# Autodesk Inventor assembly: PS20025
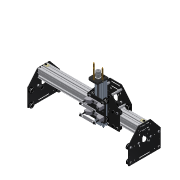
[picture p0: Inventor's stored thumbnail of the model, 180x180]
Saved by Autodesk Inventor 2014 (Build 180170000, 170)
## iProperties
Created: 2013-09-18
Part Number: PS20025
Document SubType Name: Assembly
Designer: Edward
Description: Complete Gantry
Author: Edward
Title: Complete Gantry
Subject: Shapeoko 2
## Documents named in this file (9)
- C:\Users\Edward\Documents\GitHub\Shapeoko_2\Autodesk_Inventor_Project\PS20025.iam
- C:\Users\Edward\Documents\GitHub\Shapeoko_2\Autodesk_Inventor_Project\PS20031.iam
- C:\Users\Edward\Documents\GitHub\Shapeoko_2\Autodesk_Inventor_Project\PS20008.ipt
- C:\Users\Edward\Documents\GitHub\Shapeoko_2\Autodesk_Inventor_Project\PS20022.iam
- C:\Users\Edward\Documents\GitHub\Shapeoko_2\Autodesk_Inventor_Project\25286-02.ipt
- C:\Users\Edward\Documents\GitHub\Shapeoko_2\Autodesk_Inventor_Project\25287-02.ipt
- C:\Users\Edward\Documents\GitHub\Shapeoko_2\Autodesk_Inventor_Project\26051-01.ipt
- C:\Users\Edward\Documents\GitHub\Shapeoko_2\Autodesk_Inventor_Project\PS20003.ipt
- C:\Users\Edward\Documents\GitHub\Shapeoko_2\Autodesk_Inventor_Project\26016-01.ipt
## Components (29 placed, 8 different names)
1. PS20031:1 [sub-assembly] — Mate:1, Flush:1, Mate:2, Flush:2
2. PS20022:2 [sub-assembly] — Insert:2, Insert:3, Mate:10
3. PS20008:2 — Mate:1, Flush:1, Flush:3, Insert:2, Insert:3, Mate:3, Insert:4, Insert:5, Insert:6, Insert:10, Insert:14, Insert:16
4. 25286-02:1
5. 25287-02:1 — Insert:6
6. PS20008:3 — Mate:2, Flush:2, Flush:3, Insert:11, Insert:12, Insert:18, Insert:20, Mate:7, Mate:9
7. PS20022:3 [sub-assembly] — Mate:3, Insert:4, Insert:5, Mate:8
8. 25286-02:2
9. 25287-02:2 — Insert:12
10. 25286-02:3
11. 25287-02:3 — Insert:11
12. 25286-02:4
13. 25287-02:4 — Insert:10
14. 25286-02:5
15. 25287-02:5 — Insert:14
16. 25286-02:6
17. 25287-02:6 — Insert:16
18. 25286-02:7
19. 25287-02:7 — Insert:18
20. 25286-02:8
21. 25287-02:8 — Insert:20
22. 26051-01:1 — Mate:7, Mate:8
23. PS20003:1
24. 25287-02:9
25. 26016-01:1
26. 26051-01:2 — Mate:9, Mate:10
27. PS20003:2
28. 25287-02:10
29. 26016-01:2
## Relationships (38: Insert 26, Mate 7, Flush 3, Angle 2)
- [Insert]: 25286-02:1 ↔ 25287-02:1
- Mate:1 (6.35 mm): PS20031:1 ↔ PS20008:2
- Flush:1 (25 mm): PS20031:1 ↔ PS20008:2
- Mate:2 (6.35 mm): PS20031:1 ↔ PS20008:3
- Flush:2 (25 mm): PS20031:1 ↔ PS20008:3
- Flush:3: PS20008:2 ↔ PS20008:3
- Insert:2: PS20022:2 ↔ PS20008:2
- Insert:3: PS20022:2 ↔ PS20008:2
- Mate:3: PS20008:2 ↔ PS20022:3
- Insert:4: PS20008:2 ↔ PS20022:3
- Insert:5: PS20008:2 ↔ PS20022:3
- Insert:6 (3.4163 mm): PS20008:2 ↔ 25287-02:1
- [Insert]: 25286-02:2 ↔ 25287-02:2
- [Insert]: 25286-02:3 ↔ 25287-02:3
- [Insert]: 25286-02:4 ↔ 25287-02:4
- Insert:10 (3.4163 mm): PS20008:2 ↔ 25287-02:4
- Insert:11 (3.4163 mm): PS20008:3 ↔ 25287-02:3
- Insert:12 (3.4163 mm): PS20008:3 ↔ 25287-02:2
- [Insert]: 25286-02:5 ↔ 25287-02:5
- Insert:14 (3.4163 mm): PS20008:2 ↔ 25287-02:5
- [Insert]: 25286-02:6 ↔ 25287-02:6
- Insert:16 (3.4163 mm): PS20008:2 ↔ 25287-02:6
- [Insert]: 25286-02:7 ↔ 25287-02:7
- Insert:18 (3.4163 mm): PS20008:3 ↔ 25287-02:7
- [Insert]: 25286-02:8 ↔ 25287-02:8
- Insert:20 (3.4163 mm): PS20008:3 ↔ 25287-02:8
- [Insert]: PS20003:1 ↔ 25287-02:9
- [Insert]: 26051-01:1 ↔ 25287-02:9
- [Insert] (3 mm): 26051-01:1 ↔ 26016-01:1
- [Angle] (0 deg): 26051-01:1 ↔ 26016-01:1
- Mate:7: PS20008:3 ↔ 26051-01:1
- Mate:8: PS20022:3 ↔ 26051-01:1
- [Insert]: PS20003:2 ↔ 25287-02:10
- [Insert]: 26051-01:2 ↔ 25287-02:10
- [Insert] (3 mm): 26051-01:2 ↔ 26016-01:2
- [Angle] (0 deg): 26051-01:2 ↔ 26016-01:2
- Mate:9: PS20008:3 ↔ 26051-01:2
- Mate:10: PS20022:2 ↔ 26051-01:2
## Named parameters: d101_d55_d51 = 0 mm, d20_d101_d55_d51 = 0 mm, d21_d101_d55_d51 = 0 mm, d22_d101_d55_d51 = 0 mm, d26_d101_d55_d51 = 0 mm, d28_d101_d55_d51 = 0 mm, d30_d101_d55_d51 = 0 mm, d32_d101_d55_d51 = 0 mm, d44_d0 = 0 mm, d45_d1 = 0 mm, d46_d2 = 3 mm, d47_d3 = 0 deg
